# Autodesk Inventor assembly: robot_RLRLR
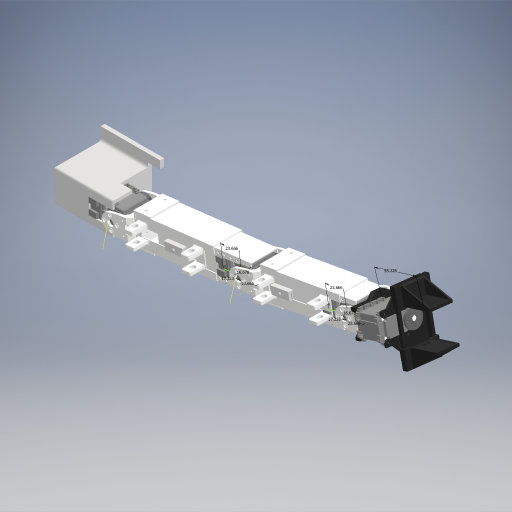
[picture p0: Inventor's stored thumbnail of the model, 512x512]
Saved by Autodesk Inventor 2024 (Build 280153000, 153)
## iProperties
Created: 2023-09-03
Part Number: robot_RLRLR
Document SubType Name: Assembly
Designer: arrusr01
Author: arrusr01
## Documents named in this file (5)
- C:\Users\arrusr01\OneDrive\Semestres\Inventor\Adaptable\robot_RLRLR.iam
- C:\Users\arrusr01\OneDrive\Semestres\Inventor\Adaptable\Base.iam
- C:\Users\arrusr01\OneDrive\Semestres\Inventor\Adaptable\Eslabon_motor_R.iam
- C:\Users\arrusr01\OneDrive\Semestres\Inventor\Adaptable\Eslabon_motor_L.iam
- C:\Users\arrusr01\OneDrive\Semestres\Inventor\Adaptable\Gripper.iam
## Components (6 placed, 4 different names)
1. Base:1 [sub-assembly] — Rotational:1
2. Eslabon_motor_R:1 [sub-assembly] — Rotational:1, Mate:1, Mate:2
3. Eslabon_motor_L:1 [sub-assembly] — Mate:1, Mate:2, Rotational:2
4. Eslabon_motor_R:2 [sub-assembly] — Rotational:2, Mate:3, Mate:4
5. Eslabon_motor_L:2 [sub-assembly] — Mate:3, Mate:4, Rotational:3
6. Gripper:1 [sub-assembly] — Rotational:3
## Relationships (7: Mate 4, RevoluteJoint 3)
- Rotational:1 [RevoluteJoint]: Base:1 ↔ Eslabon_motor_R:1
- Mate:1: Eslabon_motor_R:1 ↔ Eslabon_motor_L:1
- Mate:2: Eslabon_motor_R:1 ↔ Eslabon_motor_L:1
- Rotational:2 [RevoluteJoint]: Eslabon_motor_L:1 ↔ Eslabon_motor_R:2
- Mate:3: Eslabon_motor_R:2 ↔ Eslabon_motor_L:2
- Mate:4: Eslabon_motor_R:2 ↔ Eslabon_motor_L:2
- Rotational:3 [RevoluteJoint]: Eslabon_motor_L:2 ↔ Gripper:1
